# Autodesk Inventor assembly: Assy_foot
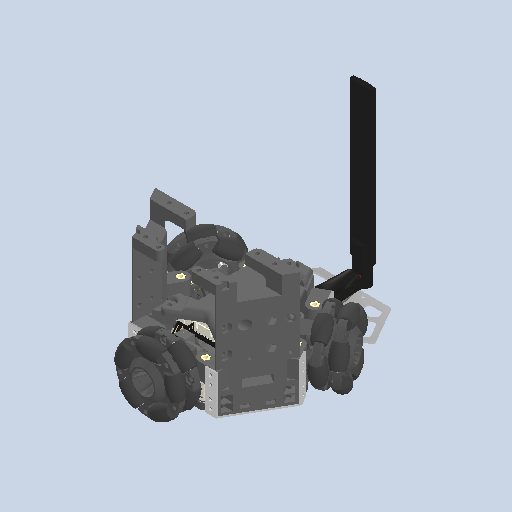
[picture p0: Inventor's stored thumbnail of the model, 512x512]
Saved by Autodesk Inventor 2024.1 (Build 281209000, 209)
## iProperties
Created: 2025-02-03
Part Number: Assy_foot
Document SubType Name: Assembly
Designer: hibik
Author: hibik
## Documents named in this file (3)
- C:\Users\hibik\Documents\Robomech\RESCUE\ORCA\hard\Assy_foot.iam
- C:\Users\hibik\Documents\Robomech\RESCUE\ORCA\hard\flame_base\base.iam
- C:\Users\hibik\Documents\Robomech\RESCUE\ORCA\hard\omni_wheel\Assy_omni_wheel.iam
## Components (4 placed, 2 different names)
1. base:1 [sub-assembly] — 挿入:1, 挿入:2, 挿入:3, 角度:1, 角度:2, 角度:3
2. Assy_omni_wheel:1 [sub-assembly] — 挿入:1, 角度:1
3. Assy_omni_wheel:2 [sub-assembly] — 挿入:2, 角度:2
4. Assy_omni_wheel:3 [sub-assembly] — 挿入:3, 角度:3
## Relationships (6: Insert 3, Angle 3)
- 挿入:1 [Insert]: base:1 ↔ Assy_omni_wheel:1
- 挿入:2 [Insert]: base:1 ↔ Assy_omni_wheel:2
- 挿入:3 [Insert]: base:1 ↔ Assy_omni_wheel:3
- 角度:1 [Angle] (0 deg): base:1 ↔ Assy_omni_wheel:1
- 角度:2 [Angle] (0 deg): base:1 ↔ Assy_omni_wheel:2
- 角度:3 [Angle] (0 deg): base:1 ↔ Assy_omni_wheel:3
